# Autodesk Inventor assembly: Forarm Assembly
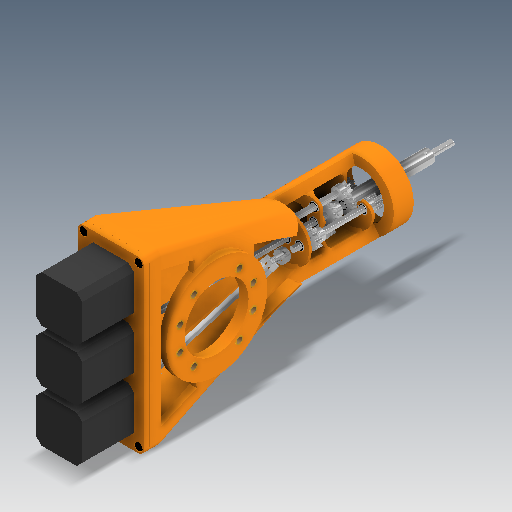
[picture p0: Inventor's stored thumbnail of the model, 512x512]
Saved by Autodesk Inventor 2020 (Build 240168000, 168)
## iProperties
Created: 2021-07-18
Part Number: Forarm Assembly
Document SubType Name: Assembly
Designer: Coy
Author: Coy
## Documents named in this file (21)
- E:\Documents\3D Files\Project 3D Models\Industrial 6 Axis Robot Arm\4th 5th amd 6th axis model\V2\Assemblys\KR500 Forarm Assembly.iam
- E:\Documents\3D Files\Project 3D Models\Industrial 6 Axis Robot Arm\4th 5th amd 6th axis model\V2\Forarm Frame.ipt
- E:\Documents\3D Files\Project 3D Models\Industrial 6 Axis Robot Arm\4th 5th amd 6th axis model\V2\Forarm Motor Mounting Plate.ipt
- E:\Documents\3D Files\Project 3D Models\Industrial 6 Axis Robot Arm\4th 5th amd 6th axis model\V2\Bearings\5mm ID 8mm OD 2.5mm Deep Roller Bearing.ipt
- E:\Documents\3D Files\Project 3D Models\Industrial 6 Axis Robot Arm\4th 5th amd 6th axis model\V2\Nema 17 Stepper Motor.ipt
- E:\Documents\3D Files\Project 3D Models\Industrial 6 Axis Robot Arm\4th 5th amd 6th axis model\V2\Gears and Couplers\5x24mm Universal Joint\Assembly.iam
- E:\Documents\3D Files\Project 3D Models\Industrial 6 Axis Robot Arm\4th 5th amd 6th axis model\V2\Shafts and Rods\M5 D Profile Rotary Shaft 47mm.ipt
- E:\Documents\3D Files\Project 3D Models\Industrial 6 Axis Robot Arm\4th 5th amd 6th axis model\V2\Gears and Couplers\5mm D Profile Coupler.ipt
- E:\Documents\3D Files\Project 3D Models\Industrial 6 Axis Robot Arm\4th 5th amd 6th axis model\V2\M12 Hollow Shaft With 12 Tooth Helical Gear.ipt
- E:\Documents\3D Files\Project 3D Models\Industrial 6 Axis Robot Arm\4th 5th amd 6th axis model\V2\Gears and Couplers\M5 6 Tooth D Profile Helical Drive Gear.ipt
- E:\Documents\3D Files\Project 3D Models\Industrial 6 Axis Robot Arm\4th 5th amd 6th axis model\V2\Gears and Couplers\M5 7 Tooth D Profile Spur Drive Gear.ipt
- E:\Documents\3D Files\Project 3D Models\Industrial 6 Axis Robot Arm\4th 5th amd 6th axis model\V2\Gears and Couplers\M5 10 Tooth D Profile Spur Drive Gear.ipt
- E:\Documents\3D Files\Project 3D Models\Industrial 6 Axis Robot Arm\4th 5th amd 6th axis model\V2\Gears and Couplers\M5 12 Tooth D Profile Helical Drive Gear.ipt
- E:\Documents\3D Files\Project 3D Models\Industrial 6 Axis Robot Arm\4th 5th amd 6th axis model\V2\Nuts and Bolts\M4 6mm OD 6mm Deep Threaded Insert.ipt
- E:\Documents\3D Files\Project 3D Models\Industrial 6 Axis Robot Arm\4th 5th amd 6th axis model\V2\Nuts and Bolts\M4 x 8 Socket Head Bolt.ipt
- E:\Documents\3D Files\Project 3D Models\Industrial 6 Axis Robot Arm\4th 5th amd 6th axis model\V2\Nuts and Bolts\M5 7mm OD 6mm Deep Threaded Insert.ipt
- E:\Documents\3D Files\Project 3D Models\Industrial 6 Axis Robot Arm\4th 5th amd 6th axis model\V2\Shafts and Rods\M5 D Profile Rotary Shaft 62mm.ipt
- E:\Documents\3D Files\Project 3D Models\Industrial 6 Axis Robot Arm\4th 5th amd 6th axis model\V2\Shafts and Rods\M5 D Profile Rotary Shaft 165mm.ipt
- E:\Documents\3D Files\Project 3D Models\Industrial 6 Axis Robot Arm\4th 5th amd 6th axis model\V2\Shafts and Rods\M5 D Profile Rotary Shaft 78mm.ipt
- E:\Documents\3D Files\Project 3D Models\Industrial 6 Axis Robot Arm\4th 5th amd 6th axis model\V2\Shafts and Rods\M5 D Profile Rotary Shaft 109mm.ipt
- E:\Documents\3D Files\Project 3D Models\Industrial 6 Axis Robot Arm\4th 5th amd 6th axis model\V2\Shafts and Rods\M5 D Profile Rotary Shaft 123mm.ipt
## Components (56 placed, 20 different names)
1. Forarm Frame:1 — Mate:6, Flush:6, Mate:10, Flush:10, Mate:11, Flush:11, Mate:12, Flush:12, Mate:13, Mate:14, Mate:15, Mate:49, Flush:25, Mate:50, Flush:26, Mate:59, Flush:32, Mate:60, Flush:33, Mate:61, Flush:34, Mate:62, Flush:35, Mate:71, Mate:72, Mate:73, Mate:74, Mate:75, Mate:76, Mate:77, Mate:78, Flush:36, Flush:37, Flush:38, Flush:39, Flush:40, Flush:41, Flush:42, Flush:43, Mate:80, Flush:44, Mate:81, Flush:45, Mate:82, Flush:46, Mate:83, Flush:47, Mate:84, Flush:48, Mate:89, Flush:49, Mate:105, Mate:111, Mate:113
2. Forarm Motor Mounting Plate:1 — Mate:13, Mate:14, Mate:15, Mate:16, Mate:17, Mate:18, Mate:19, Mate:20, Mate:21, Angle:1, Angle:2, Angle:3, Mate:63, Mate:64, Mate:65, Mate:66, Mate:67, Mate:68, Mate:69, Mate:70
3. 5mm ID 8mm OD 2.5mm Deep Roller Bearing:1 — Mate:83, Flush:47
4. 5mm ID 8mm OD 2.5mm Deep Roller Bearing:2 — Mate:81, Flush:45, Mate:106
5. 5mm ID 8mm OD 2.5mm Deep Roller Bearing:3 — Mate:6, Flush:6, Mate:94
6. 5mm ID 8mm OD 2.5mm Deep Roller Bearing:4 — Mate:80, Flush:44
7. 5mm ID 8mm OD 2.5mm Deep Roller Bearing:6 — Mate:84, Flush:48, Mate:107
8. 5mm ID 8mm OD 2.5mm Deep Roller Bearing:7 — Mate:10, Flush:10, Mate:102
9. 5mm ID 8mm OD 2.5mm Deep Roller Bearing:8 — Mate:82, Flush:46
10. 5mm ID 8mm OD 2.5mm Deep Roller Bearing:10 — Mate:12, Flush:12, Mate:122
11. 5mm ID 8mm OD 2.5mm Deep Roller Bearing:11 — Mate:11, Flush:11
12. Nema 17 Stepper Motor:1 — Mate:16, Mate:19, Angle:1, Mate:27, Flush:17
13. Nema 17 Stepper Motor:2 — Mate:17, Mate:20, Angle:2, Mate:32, Mate:33, Mate:96
14. Nema 17 Stepper Motor:3 — Mate:18, Mate:21, Angle:3, Mate:23, Flush:14
15. Assembly:1 [sub-assembly] — Mate:23, Flush:14, Mate:115, Flush:56
16. Assembly:2 [sub-assembly] — Mate:114, Flush:55, Mate:116
17. Assembly:3 [sub-assembly] — Mate:117, Flush:57, Mate:119
18. Assembly:4 [sub-assembly] — Mate:27, Flush:17, Flush:58, Mate:118
19. 5mm D Profile Coupler:1 — Mate:32, Mate:33, Mate:97
20. M12 Hollow Shaft With 12 Tooth Helical Gear:1 — Mate:38, Flush:23, Mate:39, Flush:24, Rotation:13, Mate:89, Flush:50
21. 5mm ID 8mm OD 2.5mm Deep Roller Bearing:12 — Mate:39, Flush:24, Mate:120
22. 5mm ID 8mm OD 2.5mm Deep Roller Bearing:13 — Mate:38, Flush:23
23. M5 6 Tooth D Profile Helical Drive Gear:1 — Mate:93, Mate:95, Flush:50
24. M5 6 Tooth D Profile Helical Drive Gear:2 — Rotation:13, Mate:103, Flush:52
25. M5 7 Tooth D Profile Spur Drive Gear:1 — Mate:55, Mate:104, Mate:105
26. M5 7 Tooth D Profile Spur Drive Gear:2 — Mate:110, Mate:111
27. M5 7 Tooth D Profile Spur Drive Gear:3 — Mate:112, Mate:113
28. M5 10 Tooth D Profile Spur Drive Gear:1 — Mate:55, Flush:29, Mate:108
29. M5 10 Tooth D Profile Spur Drive Gear:2 — Flush:29, Mate:109
30. M5 12 Tooth D Profile Helical Drive Gear:1 — Mate:93, Mate:123
31. 5mm ID 8mm OD 2.5mm Deep Roller Bearing:14 — Mate:49, Flush:25
32. 5mm ID 8mm OD 2.5mm Deep Roller Bearing:15 — Mate:50, Flush:26
33. M4 6mm OD 6mm Deep Threaded Insert:1 — Mate:60, Flush:33
34. M4 6mm OD 6mm Deep Threaded Insert:2 — Mate:62, Flush:35
35. M4 6mm OD 6mm Deep Threaded Insert:3 — Mate:59, Flush:32
36. M4 6mm OD 6mm Deep Threaded Insert:4 — Mate:61, Flush:34
37. M4 x 8 Socket Head Bolt:1 — Mate:63, Mate:67
38. M4 x 8 Socket Head Bolt:2 — Mate:65, Mate:70
39. M4 x 8 Socket Head Bolt:3 — Mate:64, Mate:68
40. M4 x 8 Socket Head Bolt:4 — Mate:66, Mate:69
41. M5 7mm OD 6mm Deep Threaded Insert:1 — Mate:74, Flush:40
42. M5 7mm OD 6mm Deep Threaded Insert:2 — Mate:73, Flush:39
43. M5 7mm OD 6mm Deep Threaded Insert:3 — Mate:71, Flush:37
44. M5 7mm OD 6mm Deep Threaded Insert:4 — Mate:75, Flush:41
45. M5 7mm OD 6mm Deep Threaded Insert:5 — Mate:76, Flush:42
46. M5 7mm OD 6mm Deep Threaded Insert:6 — Mate:72, Flush:38
47. M5 7mm OD 6mm Deep Threaded Insert:7 — Mate:78, Flush:36
48. M5 7mm OD 6mm Deep Threaded Insert:8 — Mate:77, Flush:43
49. M5 D Profile Rotary Shaft 62mm:1 — Mate:94, Flush:49, Mate:95, Flush:51, Flush:54, Mate:114, Flush:55
50. M5 D Profile Rotary Shaft 165mm:1 — Mate:96, Mate:97, Mate:104, Mate:121
51. M5 D Profile Rotary Shaft 47mm:1 — Mate:102, Flush:51, Mate:103, Flush:52, Flush:53, Mate:117, Flush:57
52. M5 D Profile Rotary Shaft 78mm:1 — Mate:107, Flush:54, Mate:109, Mate:110
53. M5 D Profile Rotary Shaft 78mm:2 — Mate:106, Flush:53, Mate:108, Mate:112
54. M5 D Profile Rotary Shaft 109mm:1 — Mate:115, Flush:56, Mate:116
55. M5 D Profile Rotary Shaft 109mm:2 — Flush:58, Mate:118, Mate:119
56. M5 D Profile Rotary Shaft 123mm:1 — Mate:120, Mate:121, Mate:122, Mate:123
## Relationships (117: Mate 75, Flush 38, Angle 3, RelateRotation 1)
- Mate:6: Forarm Frame:1 ↔ 5mm ID 8mm OD 2.5mm Deep Roller Bearing:3
- Flush:6: Forarm Frame:1 ↔ 5mm ID 8mm OD 2.5mm Deep Roller Bearing:3
- Mate:10: Forarm Frame:1 ↔ 5mm ID 8mm OD 2.5mm Deep Roller Bearing:7
- Flush:10: Forarm Frame:1 ↔ 5mm ID 8mm OD 2.5mm Deep Roller Bearing:7
- Mate:11: Forarm Frame:1 ↔ 5mm ID 8mm OD 2.5mm Deep Roller Bearing:11
- Flush:11: Forarm Frame:1 ↔ 5mm ID 8mm OD 2.5mm Deep Roller Bearing:11
- Mate:12: Forarm Frame:1 ↔ 5mm ID 8mm OD 2.5mm Deep Roller Bearing:10
- Flush:12: Forarm Frame:1 ↔ 5mm ID 8mm OD 2.5mm Deep Roller Bearing:10
- Mate:13: Forarm Frame:1 ↔ Forarm Motor Mounting Plate:1
- Mate:14: Forarm Frame:1 ↔ Forarm Motor Mounting Plate:1
- Mate:15 (0.1 mm): Forarm Frame:1 ↔ Forarm Motor Mounting Plate:1
- Mate:16: Forarm Motor Mounting Plate:1 ↔ Nema 17 Stepper Motor:1
- Mate:17: Forarm Motor Mounting Plate:1 ↔ Nema 17 Stepper Motor:2
- Mate:18: Forarm Motor Mounting Plate:1 ↔ Nema 17 Stepper Motor:3
- Mate:19 (0.1 mm): Forarm Motor Mounting Plate:1 ↔ Nema 17 Stepper Motor:1
- Mate:20 (0.1 mm): Forarm Motor Mounting Plate:1 ↔ Nema 17 Stepper Motor:2
- Mate:21 (0.1 mm): Forarm Motor Mounting Plate:1 ↔ Nema 17 Stepper Motor:3
- Angle:1 (0 deg): Forarm Motor Mounting Plate:1 ↔ Nema 17 Stepper Motor:1
- Angle:2 (0 deg): Forarm Motor Mounting Plate:1 ↔ Nema 17 Stepper Motor:2
- Angle:3 (0 deg): Forarm Motor Mounting Plate:1 ↔ Nema 17 Stepper Motor:3
- Mate:23: Nema 17 Stepper Motor:3 ↔ Assembly:1
- Flush:14: Nema 17 Stepper Motor:3 ↔ Assembly:1
- Mate:27: Nema 17 Stepper Motor:1 ↔ Assembly:4
- Flush:17: Nema 17 Stepper Motor:1 ↔ Assembly:4
- Mate:32: Nema 17 Stepper Motor:2 ↔ 5mm D Profile Coupler:1
- Mate:33 (-6 mm): Nema 17 Stepper Motor:2 ↔ 5mm D Profile Coupler:1
- Mate:38: M12 Hollow Shaft With 12 Tooth Helical Gear:1 ↔ 5mm ID 8mm OD 2.5mm Deep Roller Bearing:13
- Flush:23: M12 Hollow Shaft With 12 Tooth Helical Gear:1 ↔ 5mm ID 8mm OD 2.5mm Deep Roller Bearing:13
- Mate:39: M12 Hollow Shaft With 12 Tooth Helical Gear:1 ↔ 5mm ID 8mm OD 2.5mm Deep Roller Bearing:12
- Flush:24: M12 Hollow Shaft With 12 Tooth Helical Gear:1 ↔ 5mm ID 8mm OD 2.5mm Deep Roller Bearing:12
- Mate:49: Forarm Frame:1 ↔ 5mm ID 8mm OD 2.5mm Deep Roller Bearing:14
- Flush:25: Forarm Frame:1 ↔ 5mm ID 8mm OD 2.5mm Deep Roller Bearing:14
- Mate:50: Forarm Frame:1 ↔ 5mm ID 8mm OD 2.5mm Deep Roller Bearing:15
- Flush:26: Forarm Frame:1 ↔ 5mm ID 8mm OD 2.5mm Deep Roller Bearing:15
- Mate:55 (-5.5 mm): M5 7 Tooth D Profile Spur Drive Gear:1 ↔ M5 10 Tooth D Profile Spur Drive Gear:1
- Flush:29: M5 10 Tooth D Profile Spur Drive Gear:1 ↔ M5 10 Tooth D Profile Spur Drive Gear:2
- Rotation:13 [RelateRotation] (0.5 ul): M12 Hollow Shaft With 12 Tooth Helical Gear:1 ↔ M5 6 Tooth D Profile Helical Drive Gear:2
- Mate:59: Forarm Frame:1 ↔ M4 6mm OD 6mm Deep Threaded Insert:3
- Flush:32: Forarm Frame:1 ↔ M4 6mm OD 6mm Deep Threaded Insert:3
- Mate:60: Forarm Frame:1 ↔ M4 6mm OD 6mm Deep Threaded Insert:1
- Flush:33: Forarm Frame:1 ↔ M4 6mm OD 6mm Deep Threaded Insert:1
- Mate:61: Forarm Frame:1 ↔ M4 6mm OD 6mm Deep Threaded Insert:4
- Flush:34: Forarm Frame:1 ↔ M4 6mm OD 6mm Deep Threaded Insert:4
- Mate:62: Forarm Frame:1 ↔ M4 6mm OD 6mm Deep Threaded Insert:2
- Flush:35: Forarm Frame:1 ↔ M4 6mm OD 6mm Deep Threaded Insert:2
- Mate:63: Forarm Motor Mounting Plate:1 ↔ M4 x 8 Socket Head Bolt:1
- Mate:64: Forarm Motor Mounting Plate:1 ↔ M4 x 8 Socket Head Bolt:3
- Mate:65: Forarm Motor Mounting Plate:1 ↔ M4 x 8 Socket Head Bolt:2
- Mate:66: Forarm Motor Mounting Plate:1 ↔ M4 x 8 Socket Head Bolt:4
- Mate:67: Forarm Motor Mounting Plate:1 ↔ M4 x 8 Socket Head Bolt:1
- Mate:68: Forarm Motor Mounting Plate:1 ↔ M4 x 8 Socket Head Bolt:3
- Mate:69: Forarm Motor Mounting Plate:1 ↔ M4 x 8 Socket Head Bolt:4
- Mate:70: Forarm Motor Mounting Plate:1 ↔ M4 x 8 Socket Head Bolt:2
- Mate:71: Forarm Frame:1 ↔ M5 7mm OD 6mm Deep Threaded Insert:3
- Mate:72: Forarm Frame:1 ↔ M5 7mm OD 6mm Deep Threaded Insert:6
- Mate:73: Forarm Frame:1 ↔ M5 7mm OD 6mm Deep Threaded Insert:2
- Mate:74: Forarm Frame:1 ↔ M5 7mm OD 6mm Deep Threaded Insert:1
- Mate:75: Forarm Frame:1 ↔ M5 7mm OD 6mm Deep Threaded Insert:4
- Mate:76: Forarm Frame:1 ↔ M5 7mm OD 6mm Deep Threaded Insert:5
- Mate:77: Forarm Frame:1 ↔ M5 7mm OD 6mm Deep Threaded Insert:8
- Mate:78: Forarm Frame:1 ↔ M5 7mm OD 6mm Deep Threaded Insert:7
- Flush:36: Forarm Frame:1 ↔ M5 7mm OD 6mm Deep Threaded Insert:7
- Flush:37: Forarm Frame:1 ↔ M5 7mm OD 6mm Deep Threaded Insert:3
- Flush:38: Forarm Frame:1 ↔ M5 7mm OD 6mm Deep Threaded Insert:6
- Flush:39: Forarm Frame:1 ↔ M5 7mm OD 6mm Deep Threaded Insert:2
- Flush:40: Forarm Frame:1 ↔ M5 7mm OD 6mm Deep Threaded Insert:1
- Flush:41: Forarm Frame:1 ↔ M5 7mm OD 6mm Deep Threaded Insert:4
- Flush:42: Forarm Frame:1 ↔ M5 7mm OD 6mm Deep Threaded Insert:5
- Flush:43: Forarm Frame:1 ↔ M5 7mm OD 6mm Deep Threaded Insert:8
- Mate:80: Forarm Frame:1 ↔ 5mm ID 8mm OD 2.5mm Deep Roller Bearing:4
- Flush:44: Forarm Frame:1 ↔ 5mm ID 8mm OD 2.5mm Deep Roller Bearing:4
- Mate:81: Forarm Frame:1 ↔ 5mm ID 8mm OD 2.5mm Deep Roller Bearing:2
- Flush:45: Forarm Frame:1 ↔ 5mm ID 8mm OD 2.5mm Deep Roller Bearing:2
- Mate:82: Forarm Frame:1 ↔ 5mm ID 8mm OD 2.5mm Deep Roller Bearing:8
- Flush:46: Forarm Frame:1 ↔ 5mm ID 8mm OD 2.5mm Deep Roller Bearing:8
- Mate:83: Forarm Frame:1 ↔ 5mm ID 8mm OD 2.5mm Deep Roller Bearing:1
- Flush:47: Forarm Frame:1 ↔ 5mm ID 8mm OD 2.5mm Deep Roller Bearing:1
- Mate:84: Forarm Frame:1 ↔ 5mm ID 8mm OD 2.5mm Deep Roller Bearing:6
- Flush:48: Forarm Frame:1 ↔ 5mm ID 8mm OD 2.5mm Deep Roller Bearing:6
- Mate:89 (1 mm): Forarm Frame:1 ↔ M12 Hollow Shaft With 12 Tooth Helical Gear:1
- Mate:93: M5 6 Tooth D Profile Helical Drive Gear:1 ↔ M5 12 Tooth D Profile Helical Drive Gear:1
- Mate:94: 5mm ID 8mm OD 2.5mm Deep Roller Bearing:3 ↔ M5 D Profile Rotary Shaft 62mm:1
- Flush:49 (-6 mm): Forarm Frame:1 ↔ M5 D Profile Rotary Shaft 62mm:1
- Mate:95: M5 6 Tooth D Profile Helical Drive Gear:1 ↔ M5 D Profile Rotary Shaft 62mm:1
- Flush:50 (0.5 mm): M12 Hollow Shaft With 12 Tooth Helical Gear:1 ↔ M5 6 Tooth D Profile Helical Drive Gear:1
- Mate:96: Nema 17 Stepper Motor:2 ↔ M5 D Profile Rotary Shaft 165mm:1
- Mate:97: 5mm D Profile Coupler:1 ↔ M5 D Profile Rotary Shaft 165mm:1
- Mate:102: 5mm ID 8mm OD 2.5mm Deep Roller Bearing:7 ↔ M5 D Profile Rotary Shaft 47mm:1
- Flush:51: M5 D Profile Rotary Shaft 62mm:1 ↔ M5 D Profile Rotary Shaft 47mm:1
- Mate:103: M5 6 Tooth D Profile Helical Drive Gear:2 ↔ M5 D Profile Rotary Shaft 47mm:1
- Flush:52 (-0.5 mm): M5 6 Tooth D Profile Helical Drive Gear:2 ↔ M5 D Profile Rotary Shaft 47mm:1
- Mate:104: M5 7 Tooth D Profile Spur Drive Gear:1 ↔ M5 D Profile Rotary Shaft 165mm:1
- Mate:105 (1 mm): Forarm Frame:1 ↔ M5 7 Tooth D Profile Spur Drive Gear:1
- Mate:106: 5mm ID 8mm OD 2.5mm Deep Roller Bearing:2 ↔ M5 D Profile Rotary Shaft 78mm:2
- Flush:53: M5 D Profile Rotary Shaft 47mm:1 ↔ M5 D Profile Rotary Shaft 78mm:2
- Mate:107: 5mm ID 8mm OD 2.5mm Deep Roller Bearing:6 ↔ M5 D Profile Rotary Shaft 78mm:1
- Flush:54: M5 D Profile Rotary Shaft 62mm:1 ↔ M5 D Profile Rotary Shaft 78mm:1
- Mate:108: M5 10 Tooth D Profile Spur Drive Gear:1 ↔ M5 D Profile Rotary Shaft 78mm:2
- Mate:109: M5 10 Tooth D Profile Spur Drive Gear:2 ↔ M5 D Profile Rotary Shaft 78mm:1
- Mate:110: M5 7 Tooth D Profile Spur Drive Gear:2 ↔ M5 D Profile Rotary Shaft 78mm:1
- Mate:111 (0.5 mm): Forarm Frame:1 ↔ M5 7 Tooth D Profile Spur Drive Gear:2
- Mate:112: M5 7 Tooth D Profile Spur Drive Gear:3 ↔ M5 D Profile Rotary Shaft 78mm:2
- Mate:113 (0.5 mm): Forarm Frame:1 ↔ M5 7 Tooth D Profile Spur Drive Gear:3
- Mate:114: Assembly:2 ↔ M5 D Profile Rotary Shaft 62mm:1
- Flush:55: Assembly:2 ↔ M5 D Profile Rotary Shaft 62mm:1
- Mate:115: Assembly:1 ↔ M5 D Profile Rotary Shaft 109mm:1
- Flush:56: Assembly:1 ↔ M5 D Profile Rotary Shaft 109mm:1
- Mate:116: Assembly:2 ↔ M5 D Profile Rotary Shaft 109mm:1
- Mate:117: Assembly:3 ↔ M5 D Profile Rotary Shaft 47mm:1
- Flush:57: Assembly:3 ↔ M5 D Profile Rotary Shaft 47mm:1
- Flush:58: Assembly:4 ↔ M5 D Profile Rotary Shaft 109mm:2
- Mate:118: Assembly:4 ↔ M5 D Profile Rotary Shaft 109mm:2
- Mate:119: Assembly:3 ↔ M5 D Profile Rotary Shaft 109mm:2
- Mate:120: 5mm ID 8mm OD 2.5mm Deep Roller Bearing:12 ↔ M5 D Profile Rotary Shaft 123mm:1
- Mate:121: M5 D Profile Rotary Shaft 165mm:1 ↔ M5 D Profile Rotary Shaft 123mm:1
- Mate:122: 5mm ID 8mm OD 2.5mm Deep Roller Bearing:10 ↔ M5 D Profile Rotary Shaft 123mm:1
- Mate:123: M5 12 Tooth D Profile Helical Drive Gear:1 ↔ M5 D Profile Rotary Shaft 123mm:1
